# Autodesk Inventor assembly: EL2-500
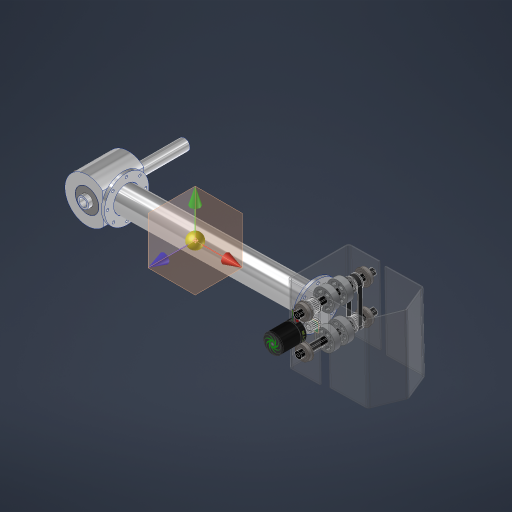
[picture p0: Inventor's stored thumbnail of the model, 512x512]
Saved by Autodesk Inventor 2023.4 (Build 274418000, 418)
## iProperties
Created: 2025-01-18
Part Number: EL2-500
Document SubType Name: Assembly
Designer: brand
Mass: 2970.22 g
Surface Area: 6958.01 cm^2
Volume: 1759.27 cm^3
Density: 1.68833 g/cm^3
Author: brand
## Documents named in this file (3)
- C:\Users\brand\OneDrive\Documents\GitHub\robotics 23\2025-ReefScape---CAD\Elevator\EL2\EL2-500.iam
- C:\Users\brand\OneDrive\Documents\GitHub\robotics 23\2025-ReefScape---CAD\Gripper\GP3\GP3-100.iam
- C:\Users\brand\OneDrive\Documents\GitHub\robotics 23\2025-ReefScape---CAD\Elevator\EL2\EL2-A-100.iam
## Components (2 placed, 2 different names)
1. EL2-A-100:1 [sub-assembly] — Insert:1, Insert:2
2. GP3-100:1 [sub-assembly] — Insert:1, Insert:2
## Relationships (2: Insert 2)
- Insert:1: EL2-A-100:1 ↔ GP3-100:1
- Insert:2: EL2-A-100:1 ↔ GP3-100:1
